# Autodesk Inventor assembly: ASY PRS 1791 top funnel 50-90_1000x90_D1200
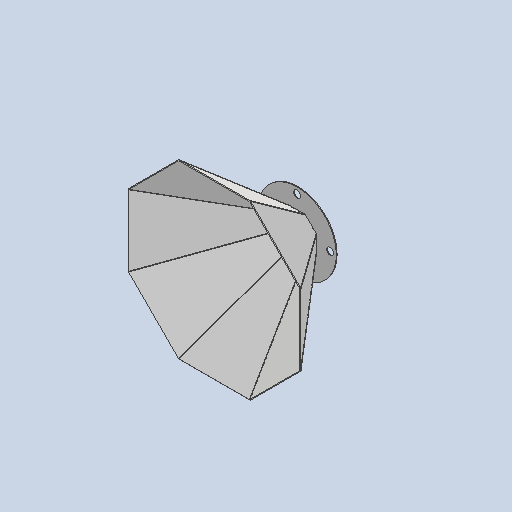
[picture p0: Inventor's stored thumbnail of the model, 512x512]
Saved by Autodesk Inventor 2026.2 (Build 302298000, 298)
## iProperties
Created: 2025-07-11
Part Number: ASY PRS 1791 top funnel 50-90_1000x90_D1200
Document SubType Name: Assembly
Designer: admin
Mass: 3988.24 g
Surface Area: 4860.23 cm^2
Volume: 498.53 cm^3
Density: 8 g/cm^3
Author: user
## Documents named in this file (3)
- C:\Users\pokla\Documents\Inventor\PRS-Purovsk\ASY PRS 1791 top funnel 50-90_1000x90_D1200.iam
- C:\Users\pokla\Documents\Inventor\PRS-Purovsk\PRS 1792 funnel FLANGE 50-90_1000x90_D1200.ipt
- C:\Users\pokla\Documents\Inventor\PRS-Purovsk\PRS 1796 top funnel 50-90_1000x90_D1200.ipt
## Components (3 placed, 2 different names)
1. PNS 1792  funnel FLANGE 1200 50-90_1000x90_1200:1 — Mate:1, Mate:2, Mate:7, Mate:3, Mate:4, Mate:6
2. PNS 1791 top funnel 1200 50-90_1000x90_1200:1 — Mate:1, Mate:2, Mate:7, Mate:5
3. PNS 1791 top funnel 1200 50-90_1000x90_1200:2 — Mate:3, Mate:4, Mate:5, Mate:6
## Relationships (7: Mate 7)
- Mate:1: PNS 1792  funnel FLANGE 1200 50-90_1000x90_1200:1 ↔ PNS 1791 top funnel 1200 50-90_1000x90_1200:1
- Mate:2: PNS 1792  funnel FLANGE 1200 50-90_1000x90_1200:1 ↔ PNS 1791 top funnel 1200 50-90_1000x90_1200:1
- Mate:7 (-2.87 mm): PNS 1792  funnel FLANGE 1200 50-90_1000x90_1200:1 ↔ PNS 1791 top funnel 1200 50-90_1000x90_1200:1
- Mate:3: PNS 1792  funnel FLANGE 1200 50-90_1000x90_1200:1 ↔ PNS 1791 top funnel 1200 50-90_1000x90_1200:2
- Mate:4: PNS 1792  funnel FLANGE 1200 50-90_1000x90_1200:1 ↔ PNS 1791 top funnel 1200 50-90_1000x90_1200:2
- Mate:5: PNS 1791 top funnel 1200 50-90_1000x90_1200:1 ↔ PNS 1791 top funnel 1200 50-90_1000x90_1200:2
- Mate:6 (-2.87 mm): PNS 1792  funnel FLANGE 1200 50-90_1000x90_1200:1 ↔ PNS 1791 top funnel 1200 50-90_1000x90_1200:2
